# Autodesk Inventor assembly: flywheel_setup
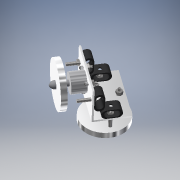
[picture p0: Inventor's stored thumbnail of the model, 180x180]
Saved by Autodesk Inventor 2017 (Build 210142000, 142)
## iProperties
Created: 2018-04-04
Part Number: flywheel_setup
Document SubType Name: Assembly
Designer: Roland
Author: Roland
## Documents named in this file (10)
- D:\Stuff\Roland\Uni\2018Sem1Courses\METR4810\progress_seminar\flywheel_setup.iam
- D:\Stuff\Roland\Uni\2018Sem1Courses\METR4810\progress_seminar\bracket_design2.ipt
- D:\Stuff\Roland\Uni\2018Sem1Courses\METR4810\progress_seminar\flywheel_design4.ipt
- D:\Stuff\Roland\Uni\2018Sem1Courses\METR4810\progress_seminar\motor_design2.ipt
- D:\Stuff\Roland\Uni\2018Sem1Courses\METR4810\progress_seminar\silicon_tube.ipt
- D:\Stuff\Roland\Uni\2018Sem1Courses\METR4810\progress_seminar\m2_bolt.ipt
- D:\Stuff\Roland\Uni\2018Sem1Courses\METR4810\progress_seminar\m2_nut.ipt
- D:\Stuff\Roland\Uni\2018Sem1Courses\METR4810\progress_seminar\m3_bolt.ipt
- D:\Stuff\Roland\Uni\2018Sem1Courses\METR4810\progress_seminar\m3_nut.ipt
- D:\Stuff\Roland\Uni\2018Sem1Courses\METR4810\progress_seminar\adapter.ipt
## Components (31 placed, 9 different names)
1. motor_design2:1 — Mate:8, Mate:9, Mate:10, Mate:25, Mate:26, Mate:27, Mate:28, Mate:29, Mate:30, Mate:64, Mate:65
2. motor_design2:2 — Mate:5, Mate:6, Mate:7, Mate:19, Mate:20, Mate:21, Mate:22, Mate:23, Mate:24, Mate:68, Mate:69, Mate:70
3. bracket_design2:1 — Mate:5, Mate:6, Mate:7, Mate:8, Mate:9, Mate:10, Mate:11, Mate:12, Angle:1, Mate:13, Mate:14, Angle:2, Mate:15, Mate:16, Angle:3, Mate:17, Mate:18, Angle:4, Mate:31, Mate:33, Mate:35, Mate:37, Mate:39, Mate:41, Mate:51, Mate:53, Mate:55, Mate:57, Mate:58, Mate:56, Mate:38, Mate:54, Mate:52, Mate:42
4. silicon_tube:1 — Mate:11, Mate:12, Angle:1, Mate:49, Mate:50
5. silicon_tube:2 — Mate:15, Mate:16, Angle:3, Mate:43, Mate:44
6. silicon_tube:3 — Mate:13, Mate:14, Angle:2, Mate:47, Mate:48
7. silicon_tube:4 — Mate:17, Mate:18, Angle:4, Mate:45, Mate:46
8. m2_bolt:1 — Mate:19, Mate:20, Mate:38, Mate:62
9. m2_bolt:2 — Mate:21, Mate:22, Mate:40
10. m2_bolt:3 — Mate:23, Mate:24, Mate:42
11. m2_bolt:4 — Mate:29, Mate:30, Mate:32
12. m2_bolt:5 — Mate:27, Mate:28, Mate:36
13. m2_bolt:6 — Mate:25, Mate:26, Mate:34
14. m2_nut:1 — Mate:31, Mate:32
15. m2_nut:2 — Mate:33, Mate:34
16. m2_nut:3 — Mate:35, Mate:36
17. m2_nut:4 — Mate:39, Mate:40
18. m2_nut:5 — Mate:41
19. m2_nut:6 — Mate:37, Mate:62
20. m3_bolt:1 — Mate:45, Mate:46, Mate:54
21. m3_bolt:2 — Mate:43, Mate:44, Mate:52
22. m3_bolt:3 — Mate:49, Mate:50, Mate:56, Mate:63
23. m3_bolt:4 — Mate:47, Mate:48, Mate:58, Mate:61
24. m3_nut:1 — Mate:51
25. m3_nut:2 — Mate:53
26. m3_nut:3 — Mate:55, Mate:63
27. m3_nut:4 — Mate:57, Mate:61
28. adapter:1 — Mate:64, Mate:65, Mate:66, Mate:67
29. adapter:2 — Mate:68, Mate:69, Mate:71
30. flywheel_design4:1 — Mate:70, Mate:71
31. flywheel_design4:2 — Mate:66, Mate:67
## Relationships (69: Mate 65, Angle 4)
- Mate:5: motor_design2:2 ↔ bracket_design2:1
- Mate:6: motor_design2:2 ↔ bracket_design2:1
- Mate:7: motor_design2:2 ↔ bracket_design2:1
- Mate:8: motor_design2:1 ↔ bracket_design2:1
- Mate:9: motor_design2:1 ↔ bracket_design2:1
- Mate:10: motor_design2:1 ↔ bracket_design2:1
- Mate:11: bracket_design2:1 ↔ silicon_tube:1
- Mate:12: bracket_design2:1 ↔ silicon_tube:1
- Angle:1 (0 deg): bracket_design2:1 ↔ silicon_tube:1
- Mate:13: bracket_design2:1 ↔ silicon_tube:3
- Mate:14: bracket_design2:1 ↔ silicon_tube:3
- Angle:2 (0 deg): bracket_design2:1 ↔ silicon_tube:3
- Mate:15: bracket_design2:1 ↔ silicon_tube:2
- Mate:16: bracket_design2:1 ↔ silicon_tube:2
- Angle:3 (0 deg): bracket_design2:1 ↔ silicon_tube:2
- Mate:17: bracket_design2:1 ↔ silicon_tube:4
- Mate:18: bracket_design2:1 ↔ silicon_tube:4
- Angle:4 (0 deg): bracket_design2:1 ↔ silicon_tube:4
- Mate:19: motor_design2:2 ↔ m2_bolt:1
- Mate:20: motor_design2:2 ↔ m2_bolt:1
- Mate:21: motor_design2:2 ↔ m2_bolt:2
- Mate:22: motor_design2:2 ↔ m2_bolt:2
- Mate:23: motor_design2:2 ↔ m2_bolt:3
- Mate:24: motor_design2:2 ↔ m2_bolt:3
- Mate:25: motor_design2:1 ↔ m2_bolt:6
- Mate:26: motor_design2:1 ↔ m2_bolt:6
- Mate:27: motor_design2:1 ↔ m2_bolt:5
- Mate:28: motor_design2:1 ↔ m2_bolt:5
- Mate:29: motor_design2:1 ↔ m2_bolt:4
- Mate:30: motor_design2:1 ↔ m2_bolt:4
- Mate:31: bracket_design2:1 ↔ m2_nut:1
- Mate:32: m2_bolt:4 ↔ m2_nut:1
- Mate:33: bracket_design2:1 ↔ m2_nut:2
- Mate:34: m2_bolt:6 ↔ m2_nut:2
- Mate:35: bracket_design2:1 ↔ m2_nut:3
- Mate:36: m2_bolt:5 ↔ m2_nut:3
- Mate:37: bracket_design2:1 ↔ m2_nut:6
- Mate:38: bracket_design2:1 ↔ m2_bolt:1
- Mate:39: bracket_design2:1 ↔ m2_nut:4
- Mate:40: m2_bolt:2 ↔ m2_nut:4
- Mate:41: bracket_design2:1 ↔ m2_nut:5
- Mate:42: bracket_design2:1 ↔ m2_bolt:3
- Mate:43: silicon_tube:2 ↔ m3_bolt:2
- Mate:44: silicon_tube:2 ↔ m3_bolt:2
- Mate:45: silicon_tube:4 ↔ m3_bolt:1
- Mate:46: silicon_tube:4 ↔ m3_bolt:1
- Mate:47: silicon_tube:3 ↔ m3_bolt:4
- Mate:48: silicon_tube:3 ↔ m3_bolt:4
- Mate:49: silicon_tube:1 ↔ m3_bolt:3
- Mate:50: silicon_tube:1 ↔ m3_bolt:3
- Mate:51: bracket_design2:1 ↔ m3_nut:1
- Mate:52: bracket_design2:1 ↔ m3_bolt:2
- Mate:53: bracket_design2:1 ↔ m3_nut:2
- Mate:54: bracket_design2:1 ↔ m3_bolt:1
- Mate:55: bracket_design2:1 ↔ m3_nut:3
- Mate:56: bracket_design2:1 ↔ m3_bolt:3
- Mate:57: bracket_design2:1 ↔ m3_nut:4
- Mate:58: bracket_design2:1 ↔ m3_bolt:4
- Mate:61: m3_bolt:4 ↔ m3_nut:4
- Mate:62: m2_bolt:1 ↔ m2_nut:6
- Mate:63: m3_bolt:3 ↔ m3_nut:3
- Mate:64: motor_design2:1 ↔ adapter:1
- Mate:65: motor_design2:1 ↔ adapter:1
- Mate:66: adapter:1 ↔ flywheel_design4:2
- Mate:67: adapter:1 ↔ flywheel_design4:2
- Mate:68: motor_design2:2 ↔ adapter:2
- Mate:69: motor_design2:2 ↔ adapter:2
- Mate:70: motor_design2:2 ↔ flywheel_design4:1
- Mate:71: adapter:2 ↔ flywheel_design4:1
